# Autodesk Inventor assembly: wyciag
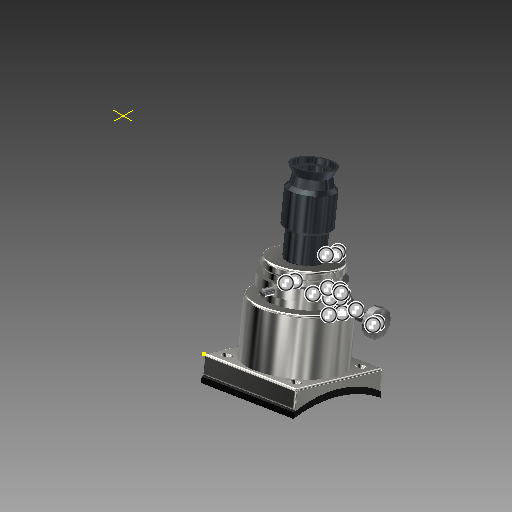
[picture p0: Inventor's stored thumbnail of the model, 512x512]
Saved by Autodesk Inventor 2019.4 (Build 234330000, 330)
## iProperties
Created: 2019-06-01
Part Number: wyciag
Document SubType Name: Assembly
Designer: Esterka
Author: Esterka
## Documents named in this file (6)
- F:\GOTOWY BEM\Wyciąg\wyciag.iam
- F:\GOTOWY BEM\Wyciąg\wyciag.ipt
- F:\GOTOWY BEM\Wyciąg\Screw GB 836 M4 x 12.ipt
- F:\GOTOWY BEM\Wyciąg\Screw GB 840 A M8 x 30.ipt
- F:\GOTOWY BEM\Wyciąg\okular.ipt
- F:\GOTOWY BEM\Wyciąg\dopasowywacz.ipt
## Components (10 placed, 5 different names)
1. wyciag:1 — Mate:3, Mate:4, Mate:5, Mate:6, Tangent:1, Tangent:2, Mate:7, Mate:8, Tangent:3, Tangent:4, Mate:9, Mate:10, Mate:11, Tangent:5, Tangent:6, Tangent:7, Zestawiające:12, Zestawiające:13
2. Screw GB/T 836-1988 M4x12:1 — Mate:10, Tangent:7
3. Screw GB/T 836-1988 M4x12:2 — Mate:9, Tangent:5
4. Screw GB/T 836-1988 M4x12:4 — Mate:11, Tangent:6
5. Screw GB/T 840-1988 Type A M8x30:1 — Mate:6, Tangent:2
6. Screw GB/T 840-1988 Type A M8x30:2 — Mate:5, Tangent:1
7. Screw GB/T 836-1988 M4x12:5 — Mate:7, Tangent:4
8. Screw GB/T 836-1988 M4x12:6 — Mate:8, Tangent:3
9. okular:1 — Mate:3, Mate:4
10. dopasowywacz:1 — Zestawiające:12, Zestawiające:13
## Relationships (18: Mate 11, Tangent 7)
- Mate:3: wyciag:1 ↔ okular:1
- Mate:4: wyciag:1 ↔ okular:1
- Mate:5: wyciag:1 ↔ Screw GB/T 840-1988 Type A M8x30:2
- Mate:6: wyciag:1 ↔ Screw GB/T 840-1988 Type A M8x30:1
- Tangent:1: wyciag:1 ↔ Screw GB/T 840-1988 Type A M8x30:2
- Tangent:2: wyciag:1 ↔ Screw GB/T 840-1988 Type A M8x30:1
- Mate:7: wyciag:1 ↔ Screw GB/T 836-1988 M4x12:5
- Mate:8: wyciag:1 ↔ Screw GB/T 836-1988 M4x12:6
- Tangent:3: wyciag:1 ↔ Screw GB/T 836-1988 M4x12:6
- Tangent:4: wyciag:1 ↔ Screw GB/T 836-1988 M4x12:5
- Mate:9: wyciag:1 ↔ Screw GB/T 836-1988 M4x12:2
- Mate:10: wyciag:1 ↔ Screw GB/T 836-1988 M4x12:1
- Mate:11: wyciag:1 ↔ Screw GB/T 836-1988 M4x12:4
- Tangent:5: wyciag:1 ↔ Screw GB/T 836-1988 M4x12:2
- Tangent:6: wyciag:1 ↔ Screw GB/T 836-1988 M4x12:4
- Tangent:7: wyciag:1 ↔ Screw GB/T 836-1988 M4x12:1
- Zestawiające:12 [Mate]: wyciag:1 ↔ dopasowywacz:1
- Zestawiające:13 [Mate]: wyciag:1 ↔ dopasowywacz:1
